# Autodesk Inventor assembly: CoreXY Motor Assembly Left for 4040 - V3
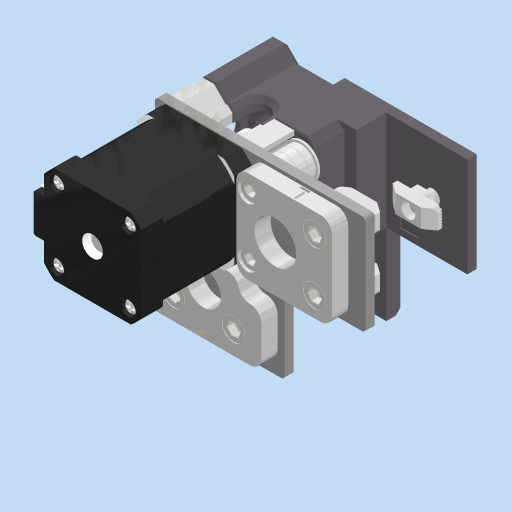
[picture p0: Inventor's stored thumbnail of the model, 512x512]
Saved by Autodesk Inventor 2023.2 (Build 272271000, 271)
## iProperties
Created: 2023-11-27
Part Number: CoreXY Motor Assembly Left for 4040 - V3
Document SubType Name: Assembly
Designer: Nils Bade
Author: Nils Bade
## Documents named in this file (18)
- C:\Users\nilsb\Documents\Inventor\Projektarbeit-Bade\RatRig_Bade\CoreXY Motor Assembly Left for 4040 - V3.iam
- C:\Users\nilsb\Documents\Inventor\Projektarbeit-Bade\RatRig_modified\Motor Plate Top for 4040.ipt
- C:\Users\nilsb\Documents\Inventor\Projektarbeit-Bade\RatRig_Standards\Nema 17 Stepper Motor - 48mm - 1.8degree_step, 76oz-in v1.ipt
- C:\Users\nilsb\Documents\Inventor\Projektarbeit-Bade\RatRig_Standards\Timing Pulley - 2GT (2mm) - 20 Tooth - For 9mm Belt - 5mm Bo v1.ipt
- C:\Users\nilsb\Documents\Inventor\Projektarbeit-Bade\Schrauben\Cap Head Screw M3x35 v2.ipt
- C:\Users\nilsb\Documents\Inventor\Projektarbeit-Bade\RatRig_modified\T-NUT - DropIn 4040 SERIES - M6.ipt
- C:\Users\nilsb\Documents\Inventor\Projektarbeit-Bade\Schrauben\Cap Head Screw M6x16.ipt
- C:\Users\nilsb\Documents\Inventor\Projektarbeit-Bade\Schrauben\Countersink Screw M6x14 v2.ipt
- C:\Users\nilsb\Documents\Inventor\Projektarbeit-Bade\Schrauben\Cap Head Screw M5x40 v2.ipt
- C:\Users\nilsb\Documents\Inventor\Projektarbeit-Bade\RatRig_Standards\Hex Locking Nut - M5 v2.ipt
- C:\Users\nilsb\Documents\Inventor\Projektarbeit-Bade\RatRig_Standards\Mini Precision Shim - 8x5x1mm v2.ipt
- C:\Users\nilsb\Documents\Inventor\Projektarbeit-Bade\RatRig_Standards\Ball Bearing - F695ZZ v1.ipt
- C:\Users\nilsb\Documents\Inventor\Projektarbeit-Bade\RatRig_Standards\Ball Bearing - 695ZZ v1.ipt
- C:\Users\nilsb\Documents\Inventor\Projektarbeit-Bade\RatRig_modified\xy Motorcage Top Left for 4040 V2.ipt
- C:\Users\nilsb\Documents\Inventor\Projektarbeit-Bade\RatRig_modified\xy Motor Support Left for 4040 V2.ipt
- C:\Users\nilsb\Documents\Inventor\Projektarbeit-Bade\RatRig_modified\xy_motor_cage_bottom_left_v4.ipt
- xy_motor_cage_bottom_left_v4.ipt
- C:\Users\nilsb\Documents\Inventor\Projektarbeit-Bade\RatRig_modified\xy Motor Support Left for 4040 extra.ipt
## Components (43 placed, 16 different names)
1. xy Motorcage Top Left for 4040 V2:2
2. xy_motor_cage_bottom_left_v4:1
3. Motor Plate Top for 4040:1 — Passend:7, Winkel:1, Passend:10, Passend:20, Passend:21, Passend:22, Passend:23, Winkel:4, Winkel:5, Winkel:8, Winkel:9, Passend:26, Passend:27, Passend:28, Passend:29, Passend:66, Passend:73, Passend:88, Passend:89, Passend:90, Passend:91, Passend:92, Passend:93, Passend:94
4. Nema 17 Stepper Motor - 48mm - 1.8degree_step, 76oz-in v1:1 — Passend:7, Winkel:1, Passend:8, Passend:9, Winkel:2, Passend:10
5. Timing Pulley - 2GT (2mm) - 20 Tooth - For 9mm Belt - 5mm Bo v1:1 — Passend:8, Passend:9, Winkel:2
6. Cap Head Screw M3x35 v2:1
7. Cap Head Screw M3x35 v2:2
8. Cap Head Screw M3x35 v2:3
9. Cap Head Screw M3x35 v2:4
10. T-NUT - DROP IN TYPE FOR 40 SERIES - M6:1 — Passend:20, Winkel:4, Passend:29
11. T-NUT - DROP IN TYPE FOR 40 SERIES - M6:2 — Passend:21, Winkel:5, Passend:28
12. T-NUT - DROP IN TYPE FOR 40 SERIES - M6:3 — Passend:23, Winkel:9, Passend:26
13. T-NUT - DROP IN TYPE FOR 40 SERIES - M6:4 — Passend:22, Winkel:8, Passend:27
14. T-NUT - DROP IN TYPE FOR 40 SERIES - M6:5
15. T-NUT - DROP IN TYPE FOR 40 SERIES - M6:6
16. T-NUT - DROP IN TYPE FOR 40 SERIES - M6:7
17. Cap Head Screw M6x16:1 — Passend:94, Passend:98
18. Cap Head Screw M6x16:2 — Passend:93, Passend:97
19. Cap Head Screw M6x16:3 — Passend:92, Passend:96
20. Cap Head Screw M6x16:4 — Passend:91, Passend:95
21. Countersink Screw M6x14 v2:1
22. Countersink Screw M6x14 v2:2
23. Countersink Screw M6x14 v2:3
24. xy Motor Support Left for 4040 V2:2 — Passend:97, Passend:98
25. Cap Head Screw M5x40 v2:1 — Passend:56, Passend:62, Passend:63, Passend:64, Passend:74, Passend:76, Passend:78, Passend:81, Passend:83, Passend:86
26. Cap Head Screw M5x40 v2:2 — Passend:57, Passend:60, Passend:61, Passend:65, Passend:69, Passend:71
27. Hex Locking Nut - M5 v2:1 — Passend:56
28. Hex Locking Nut - M5 v2:2 — Passend:57
29. Mini Precision Shim - 8x5x1mm v2:1 — Passend:60, Passend:66, Passend:67
30. Mini Precision Shim - 8x5x1mm v2:2 — Passend:61
31. Mini Precision Shim - 8x5x1mm v2:3 — Passend:62, Passend:73, Passend:75
32. Mini Precision Shim - 8x5x1mm v2:4 — Passend:63, Passend:80, Passend:82
33. Mini Precision Shim - 8x5x1mm v2:5 — Passend:64
34. Ball Bearing - F695ZZ v1:1 — Passend:86, Passend:87
35. Ball Bearing - F695ZZ v1:2 — Passend:78, Passend:79, Passend:80
36. Ball Bearing - F695ZZ v1:3 — Passend:71, Passend:72
37. Ball Bearing - F695ZZ v1:4 — Passend:81, Passend:82, Passend:84
38. Ball Bearing - F695ZZ v1:5 — Passend:74, Passend:75, Passend:77
39. Ball Bearing - F695ZZ v1:6 — Passend:65, Passend:67, Passend:70
40. Ball Bearing - 695ZZ v1:1 — Passend:69, Passend:70, Passend:72
41. Ball Bearing - 695ZZ v1:2 — Passend:76, Passend:77, Passend:79
42. Ball Bearing - 695ZZ v1:3 — Passend:83, Passend:84, Passend:87
43. xy Motor Support Left for 4040 extra:1 — Passend:88, Passend:89, Passend:90, Passend:95, Passend:96
## Relationships (99: Mate 88, Angle 11)
- [Mate]: xy Motorcage Top Left for 4040 V2:2 ↔ xy_motor_cage_bottom_left_v4:1
- [Mate]: xy Motorcage Top Left for 4040 V2:2 ↔ xy_motor_cage_bottom_left_v4:1
- [Mate]: xy Motorcage Top Left for 4040 V2:2 ↔ xy_motor_cage_bottom_left_v4:1
- [Mate]: xy_motor_cage_bottom_left_v4:1 ↔ Motor Plate Top for 4040:1
- [Mate]: xy_motor_cage_bottom_left_v4:1 ↔ Motor Plate Top for 4040:1
- [Mate]: xy_motor_cage_bottom_left_v4:1 ↔ Motor Plate Top for 4040:1
- Passend:7 [Mate]: Motor Plate Top for 4040:1 ↔ Nema 17 Stepper Motor - 48mm - 1.8degree_step, 76oz-in v1:1
- Winkel:1 [Angle] (0 deg): Motor Plate Top for 4040:1 ↔ Nema 17 Stepper Motor - 48mm - 1.8degree_step, 76oz-in v1:1
- Passend:8 [Mate]: Nema 17 Stepper Motor - 48mm - 1.8degree_step, 76oz-in v1:1 ↔ Timing Pulley - 2GT (2mm) - 20 Tooth - For 9mm Belt - 5mm Bo v1:1
- Passend:9 [Mate] (1 mm): Nema 17 Stepper Motor - 48mm - 1.8degree_step, 76oz-in v1:1 ↔ Timing Pulley - 2GT (2mm) - 20 Tooth - For 9mm Belt - 5mm Bo v1:1
- Winkel:2 [Angle] (0 deg): Nema 17 Stepper Motor - 48mm - 1.8degree_step, 76oz-in v1:1 ↔ Timing Pulley - 2GT (2mm) - 20 Tooth - For 9mm Belt - 5mm Bo v1:1
- Passend:10 [Mate]: Motor Plate Top for 4040:1 ↔ Nema 17 Stepper Motor - 48mm - 1.8degree_step, 76oz-in v1:1
- [Mate]: xy Motorcage Top Left for 4040 V2:2 ↔ Cap Head Screw M3x35 v2:4
- [Mate]: xy Motorcage Top Left for 4040 V2:2 ↔ Cap Head Screw M3x35 v2:2
- [Mate]: xy Motorcage Top Left for 4040 V2:2 ↔ Cap Head Screw M3x35 v2:1
- [Mate]: xy Motorcage Top Left for 4040 V2:2 ↔ Cap Head Screw M3x35 v2:3
- [Mate]: xy Motorcage Top Left for 4040 V2:2 ↔ Cap Head Screw M3x35 v2:2
- [Mate]: xy Motorcage Top Left for 4040 V2:2 ↔ Cap Head Screw M3x35 v2:4
- [Mate]: xy Motorcage Top Left for 4040 V2:2 ↔ Cap Head Screw M3x35 v2:1
- [Mate]: xy Motorcage Top Left for 4040 V2:2 ↔ Cap Head Screw M3x35 v2:3
- [Mate]: xy Motorcage Top Left for 4040 V2:2 ↔ T-NUT - DROP IN TYPE FOR 40 SERIES - M6:7
- Passend:20 [Mate]: Motor Plate Top for 4040:1 ↔ T-NUT - DROP IN TYPE FOR 40 SERIES - M6:1
- Passend:21 [Mate]: Motor Plate Top for 4040:1 ↔ T-NUT - DROP IN TYPE FOR 40 SERIES - M6:2
- Passend:22 [Mate]: Motor Plate Top for 4040:1 ↔ T-NUT - DROP IN TYPE FOR 40 SERIES - M6:4
- Passend:23 [Mate]: Motor Plate Top for 4040:1 ↔ T-NUT - DROP IN TYPE FOR 40 SERIES - M6:3
- [Mate]: xy Motorcage Top Left for 4040 V2:2 ↔ T-NUT - DROP IN TYPE FOR 40 SERIES - M6:5
- [Mate]: xy Motorcage Top Left for 4040 V2:2 ↔ T-NUT - DROP IN TYPE FOR 40 SERIES - M6:6
- [Angle] (0 deg): xy Motorcage Top Left for 4040 V2:2 ↔ T-NUT - DROP IN TYPE FOR 40 SERIES - M6:7
- Winkel:4 [Angle] (0 deg): Motor Plate Top for 4040:1 ↔ T-NUT - DROP IN TYPE FOR 40 SERIES - M6:1
- Winkel:5 [Angle] (0 deg): Motor Plate Top for 4040:1 ↔ T-NUT - DROP IN TYPE FOR 40 SERIES - M6:2
- [Angle] (0 deg): xy Motorcage Top Left for 4040 V2:2 ↔ T-NUT - DROP IN TYPE FOR 40 SERIES - M6:5
- [Angle] (0 deg): xy Motorcage Top Left for 4040 V2:2 ↔ T-NUT - DROP IN TYPE FOR 40 SERIES - M6:6
- Winkel:8 [Angle] (0 deg): Motor Plate Top for 4040:1 ↔ T-NUT - DROP IN TYPE FOR 40 SERIES - M6:4
- Winkel:9 [Angle] (0 deg): Motor Plate Top for 4040:1 ↔ T-NUT - DROP IN TYPE FOR 40 SERIES - M6:3
- Passend:26 [Mate] (5.5 mm): Motor Plate Top for 4040:1 ↔ T-NUT - DROP IN TYPE FOR 40 SERIES - M6:3
- Passend:27 [Mate] (5.5 mm): Motor Plate Top for 4040:1 ↔ T-NUT - DROP IN TYPE FOR 40 SERIES - M6:4
- Passend:28 [Mate] (5.5 mm): Motor Plate Top for 4040:1 ↔ T-NUT - DROP IN TYPE FOR 40 SERIES - M6:2
- Passend:29 [Mate] (5.5 mm): Motor Plate Top for 4040:1 ↔ T-NUT - DROP IN TYPE FOR 40 SERIES - M6:1
- [Mate] (5.5 mm): xy Motorcage Top Left for 4040 V2:2 ↔ T-NUT - DROP IN TYPE FOR 40 SERIES - M6:7
- [Mate] (5.5 mm): xy Motorcage Top Left for 4040 V2:2 ↔ T-NUT - DROP IN TYPE FOR 40 SERIES - M6:5
- [Mate] (5.5 mm): xy Motorcage Top Left for 4040 V2:2 ↔ T-NUT - DROP IN TYPE FOR 40 SERIES - M6:6
- [Mate]: xy Motorcage Top Left for 4040 V2:2 ↔ Countersink Screw M6x14 v2:3
- [Mate]: xy Motorcage Top Left for 4040 V2:2 ↔ Countersink Screw M6x14 v2:3
- [Mate]: xy Motorcage Top Left for 4040 V2:2 ↔ Countersink Screw M6x14 v2:1
- [Mate]: xy Motorcage Top Left for 4040 V2:2 ↔ Countersink Screw M6x14 v2:2
- [Mate]: xy Motorcage Top Left for 4040 V2:2 ↔ Countersink Screw M6x14 v2:1
- [Mate]: xy Motorcage Top Left for 4040 V2:2 ↔ Countersink Screw M6x14 v2:2
- [Mate]: Motor Plate Top for 4040:1 ↔ xy Motor Support Left for 4040 V2:2
- [Mate]: Motor Plate Top for 4040:1 ↔ xy Motor Support Left for 4040 V2:2
- [Mate]: Motor Plate Top for 4040:1 ↔ xy Motor Support Left for 4040 V2:2
- [Mate]: xy Motor Support Left for 4040 V2:2 ↔ Cap Head Screw M5x40 v2:1
- [Mate]: xy Motor Support Left for 4040 V2:2 ↔ Cap Head Screw M5x40 v2:2
- [Mate]: xy Motor Support Left for 4040 V2:2 ↔ Cap Head Screw M5x40 v2:2
- [Mate]: xy Motor Support Left for 4040 V2:2 ↔ Cap Head Screw M5x40 v2:1
- Passend:56 [Mate]: Cap Head Screw M5x40 v2:1 ↔ Hex Locking Nut - M5 v2:1
- Passend:57 [Mate]: Cap Head Screw M5x40 v2:2 ↔ Hex Locking Nut - M5 v2:2
- [Angle] (0 deg): xy Motorcage Top Left for 4040 V2:2 ↔ Hex Locking Nut - M5 v2:1
- [Angle] (0 deg): xy Motorcage Top Left for 4040 V2:2 ↔ Hex Locking Nut - M5 v2:2
- [Mate]: xy Motorcage Top Left for 4040 V2:2 ↔ Hex Locking Nut - M5 v2:2
- [Mate]: xy Motorcage Top Left for 4040 V2:2 ↔ Hex Locking Nut - M5 v2:1
- Passend:60 [Mate]: Cap Head Screw M5x40 v2:2 ↔ Mini Precision Shim - 8x5x1mm v2:1
- Passend:61 [Mate]: Cap Head Screw M5x40 v2:2 ↔ Mini Precision Shim - 8x5x1mm v2:2
- Passend:62 [Mate]: Cap Head Screw M5x40 v2:1 ↔ Mini Precision Shim - 8x5x1mm v2:3
- Passend:63 [Mate]: Cap Head Screw M5x40 v2:1 ↔ Mini Precision Shim - 8x5x1mm v2:4
- Passend:64 [Mate]: Cap Head Screw M5x40 v2:1 ↔ Mini Precision Shim - 8x5x1mm v2:5
- Passend:65 [Mate]: Cap Head Screw M5x40 v2:2 ↔ Ball Bearing - F695ZZ v1:6
- Passend:66 [Mate]: Motor Plate Top for 4040:1 ↔ Mini Precision Shim - 8x5x1mm v2:1
- Passend:67 [Mate]: Mini Precision Shim - 8x5x1mm v2:1 ↔ Ball Bearing - F695ZZ v1:6
- [Mate]: xy Motorcage Top Left for 4040 V2:2 ↔ Mini Precision Shim - 8x5x1mm v2:2
- Passend:69 [Mate]: Cap Head Screw M5x40 v2:2 ↔ Ball Bearing - 695ZZ v1:1
- Passend:70 [Mate]: Ball Bearing - F695ZZ v1:6 ↔ Ball Bearing - 695ZZ v1:1
- Passend:71 [Mate]: Cap Head Screw M5x40 v2:2 ↔ Ball Bearing - F695ZZ v1:3
- Passend:72 [Mate]: Ball Bearing - F695ZZ v1:3 ↔ Ball Bearing - 695ZZ v1:1
- Passend:73 [Mate]: Motor Plate Top for 4040:1 ↔ Mini Precision Shim - 8x5x1mm v2:3
- Passend:74 [Mate]: Cap Head Screw M5x40 v2:1 ↔ Ball Bearing - F695ZZ v1:5
- Passend:75 [Mate]: Mini Precision Shim - 8x5x1mm v2:3 ↔ Ball Bearing - F695ZZ v1:5
- Passend:76 [Mate]: Cap Head Screw M5x40 v2:1 ↔ Ball Bearing - 695ZZ v1:2
- Passend:77 [Mate]: Ball Bearing - F695ZZ v1:5 ↔ Ball Bearing - 695ZZ v1:2
- Passend:78 [Mate]: Cap Head Screw M5x40 v2:1 ↔ Ball Bearing - F695ZZ v1:2
- Passend:79 [Mate]: Ball Bearing - F695ZZ v1:2 ↔ Ball Bearing - 695ZZ v1:2
- Passend:80 [Mate]: Mini Precision Shim - 8x5x1mm v2:4 ↔ Ball Bearing - F695ZZ v1:2
- Passend:81 [Mate]: Cap Head Screw M5x40 v2:1 ↔ Ball Bearing - F695ZZ v1:4
- Passend:82 [Mate]: Mini Precision Shim - 8x5x1mm v2:4 ↔ Ball Bearing - F695ZZ v1:4
- Passend:83 [Mate]: Cap Head Screw M5x40 v2:1 ↔ Ball Bearing - 695ZZ v1:3
- Passend:84 [Mate]: Ball Bearing - F695ZZ v1:4 ↔ Ball Bearing - 695ZZ v1:3
- [Mate]: xy Motorcage Top Left for 4040 V2:2 ↔ Mini Precision Shim - 8x5x1mm v2:5
- Passend:86 [Mate]: Cap Head Screw M5x40 v2:1 ↔ Ball Bearing - F695ZZ v1:1
- Passend:87 [Mate]: Ball Bearing - F695ZZ v1:1 ↔ Ball Bearing - 695ZZ v1:3
- Passend:88 [Mate]: Motor Plate Top for 4040:1 ↔ xy Motor Support Left for 4040 extra:1
- Passend:89 [Mate]: Motor Plate Top for 4040:1 ↔ xy Motor Support Left for 4040 extra:1
- Passend:90 [Mate]: Motor Plate Top for 4040:1 ↔ xy Motor Support Left for 4040 extra:1
- Passend:91 [Mate]: Motor Plate Top for 4040:1 ↔ Cap Head Screw M6x16:4
- Passend:92 [Mate]: Motor Plate Top for 4040:1 ↔ Cap Head Screw M6x16:3
- Passend:93 [Mate]: Motor Plate Top for 4040:1 ↔ Cap Head Screw M6x16:2
- Passend:94 [Mate]: Motor Plate Top for 4040:1 ↔ Cap Head Screw M6x16:1
- Passend:95 [Mate]: Cap Head Screw M6x16:4 ↔ xy Motor Support Left for 4040 extra:1
- Passend:96 [Mate]: Cap Head Screw M6x16:3 ↔ xy Motor Support Left for 4040 extra:1
- Passend:97 [Mate]: Cap Head Screw M6x16:2 ↔ xy Motor Support Left for 4040 V2:2
- Passend:98 [Mate]: Cap Head Screw M6x16:1 ↔ xy Motor Support Left for 4040 V2:2
